# Autodesk Inventor assembly: First_Stage_SEC-Station
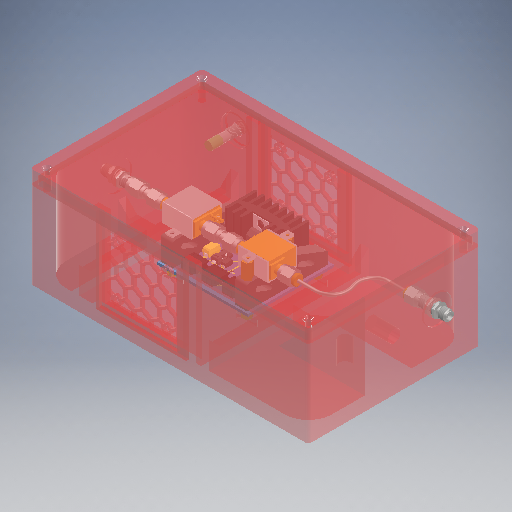
[picture p0: Inventor's stored thumbnail of the model, 512x512]
Saved by Autodesk Inventor 2025.2 (Build 292293000, 293)
## iProperties
Created: 2024-12-02
Part Number: First_Stage_SEC-Station
Document SubType Name: Assembly
Designer: Paul Linke
Author: Paul Linke
## Documents named in this file (14)
- B:\ToPush\First_Stage\First_Stage_SPIKES.iam
- B:\ToPush\First_Stage\Parts\Mini-Circuits_Package\Mini-Circuits_Package.iam
- B:\ToPush\First_Stage\Parts\Voltage_Regulator_for_ZX60-14LN-S+\Voltage_Regulator_for_ZX60-14LN-S+.iam
- B:\ToPush\First_Stage\Parts\SMA_Male-Male.ipt
- B:\ToPush\First_Stage\PCB-LNA.ipt
- B:\ToPush\First_Stage\PCB-LNA_MIR.ipt
- B:\ToPush\First_Stage\Parts\SMA_Feedthrough.ipt
- B:\ToPush\First_Stage\Parts\SMA_cable_83mm_NOiso_BENT.ipt
- B:\ToPush\First_Stage\First_Stage_BoxBottom.ipt
- B:\ToPush\First_Stage\Parts\Hex_standoff_M2.5_5mm.ipt
- B:\ToPush\First_Stage\Parts\Hex_standoff_M2.5_10mm.ipt
- B:\ToPush\First_Stage\First_Stage_HexGrill.ipt
- B:\ToPush\First_Stage\First_Stage_BoxTop.ipt
- B:\ToPush\First_Stage\Parts\FlatLED_6mm\FlatLED_6mm.iam
## Components (21 placed, 12 different names)
1. Mini-Circuits_Package:1 [sub-assembly] — Mate:7, Mate:8
2. SMA_Male-Male:1 — Mate:7, Mate:11
3. SMA_Male-Male:2 — Mate:8, Mate:9
4. Mini-Circuits_Package:2 [sub-assembly] — Mate:9, Mate:18
5. Voltage_Regulator_for_ZX60-14LN-S+:1 [sub-assembly] — Flush:1, Flush:2, Mate:10, Mate:23
6. PCB-LNA:1 — Flush:1, Flush:2
7. PCB-LNA_MIR:1 — Mate:10
8. SMA_Feedthrough:1 — Mate:11
9. SMA_Feedthrough:2 — Mate:19
10. SMA_cable_83mm_NOiso_BENT:1 — Mate:18, Mate:19
11. AS 1110 - Metric M2.5 x 6:6 — Mate:36
12. AS 1110 - Metric M2.5 x 6:11
13. AS 1110 - Metric M2.5 x 6:7
14. AS 1110 - Metric M2.5 x 6:8 — Mate:23, Mate:37
15. AS 1110 - Metric M2.5 x 6:9 — Mate:35
16. AS 1110 - Metric M2.5 x 6:10
17. First_Stage_BoxBottom:1 — Mate:31, Mate:32, Mate:33, Mate:34, Mate:35, Mate:36, Mate:37, Mate:38, Mate:39, Flush:3, Mate:40
18. First_Stage_HexGrill:2 — Mate:31, Mate:38, Mate:39
19. First_Stage_HexGrill:3 — Mate:32, Mate:33, Mate:34
20. First_Stage_BoxTop:1 — Flush:3
21. FlatLED_6mm:1 [sub-assembly] — Mate:40
## Relationships (21: Mate 18, Flush 3)
- Flush:1: Voltage_Regulator_for_ZX60-14LN-S+:1 ↔ PCB-LNA:1
- Flush:2: Voltage_Regulator_for_ZX60-14LN-S+:1 ↔ PCB-LNA:1
- Mate:7: Mini-Circuits_Package:1 ↔ SMA_Male-Male:1
- Mate:8: Mini-Circuits_Package:1 ↔ SMA_Male-Male:2
- Mate:9: SMA_Male-Male:2 ↔ Mini-Circuits_Package:2
- Mate:10: Voltage_Regulator_for_ZX60-14LN-S+:1 ↔ PCB-LNA_MIR:1
- Mate:11: SMA_Male-Male:1 ↔ SMA_Feedthrough:1
- Mate:18: Mini-Circuits_Package:2 ↔ SMA_cable_83mm_NOiso_BENT:1
- Mate:19: SMA_Feedthrough:2 ↔ SMA_cable_83mm_NOiso_BENT:1
- Mate:23: Voltage_Regulator_for_ZX60-14LN-S+:1 ↔ AS 1110 - Metric M2.5 x 6:8
- Mate:31 (0.1 mm): First_Stage_BoxBottom:1 ↔ First_Stage_HexGrill:2
- Mate:32: First_Stage_BoxBottom:1 ↔ First_Stage_HexGrill:3
- Mate:33 (0.1 mm): First_Stage_BoxBottom:1 ↔ First_Stage_HexGrill:3
- Mate:34: First_Stage_BoxBottom:1 ↔ First_Stage_HexGrill:3
- Mate:35: AS 1110 - Metric M2.5 x 6:9 ↔ First_Stage_BoxBottom:1
- Mate:36: AS 1110 - Metric M2.5 x 6:6 ↔ First_Stage_BoxBottom:1
- Mate:37: AS 1110 - Metric M2.5 x 6:8 ↔ First_Stage_BoxBottom:1
- Mate:38: First_Stage_BoxBottom:1 ↔ First_Stage_HexGrill:2
- Mate:39: First_Stage_BoxBottom:1 ↔ First_Stage_HexGrill:2
- Flush:3: First_Stage_BoxBottom:1 ↔ First_Stage_BoxTop:1
- Mate:40: First_Stage_BoxBottom:1 ↔ FlatLED_6mm:1
